# Autodesk Inventor assembly: Polea Compuesta
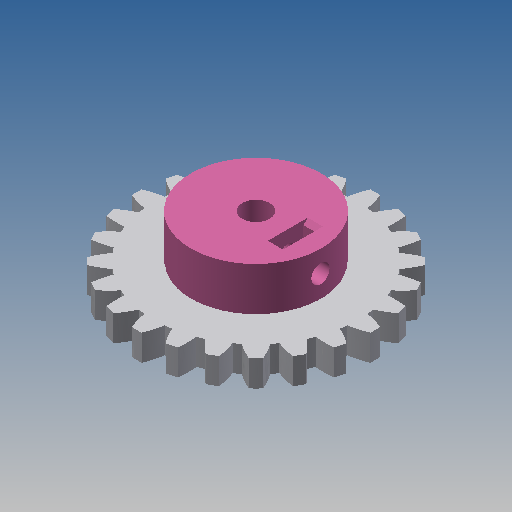
[picture p0: Inventor's stored thumbnail of the model, 512x512]
Saved by Autodesk Inventor 2017 (Build 210142000, 142)
## iProperties
Part Number: Polea Compuesta
Material: Genérico
Document SubType Name: Assembly
Designer: FABLAB
Author: FABLAB
## Documents named in this file (3)
- C:\Users\FABLAB\Documents\GitHub\actor-re-actor\models\inventor-caja\transmision Engranajes\Polea Compuesta.iam
- C:\Users\FABLAB\Documents\GitHub\actor-re-actor\models\inventor-caja\transmision Engranajes\dado polea.ipt
- C:\Users\FABLAB\Documents\GitHub\actor-re-actor\models\inventor-caja\transmision Engranajes\engrane motor-dado.ipt
## Components (2 placed, 2 different names)
1. dado polea:1 — Nivelación:1
2. engrane motor-dado:1 — Nivelación:1, Coincidencia:1, Coincidencia:2
## Relationships (3: Mate 2, Flush 1)
- Nivelación:1 [Flush]: dado polea:1 ↔ engrane motor-dado:1
- Coincidencia:1 [Mate]: engrane motor-dado:1
- Coincidencia:2 [Mate]: engrane motor-dado:1
